# Autodesk Inventor assembly: MCOCWK26-6-12
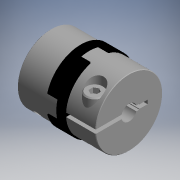
[picture p0: Inventor's stored thumbnail of the model, 180x180]
Saved by Autodesk Inventor 2017.3 (Build 213256000, 256)
## iProperties
Category: PARTsolutions
Company: MISUMI
Part Number: MCOCWK26-6-12
Catalog Web Link: www.cadenas.de
Description: MCOCLK, MCOCRK, MCOCWK-Oldham Clamping Type - Key Groove Hole Type
Vendor: MISUMI
Document SubType Name: Assembly
Designer: partserver
Manufacturer: MISUMI
Mass: 13.269 g
Surface Area: 80.443 cm^2
Volume: 13.269 cm^3
Density: 1 g/cm^3
Title: MCOCWK26-6-12
Author: Cadenas PARTsolutions
Comments: Oldham Clamping Type - Key Groove Hole Type
PSOL_IDENT_0: {$CADENAS_DATA\23d-libs\misumi\metric\50_couplings\mcocwk_asmtab.prj},243 {VTYP=3D},{STYP=ASSTAB},{N
PSOL_IDENT_1: B=MCOCWK26-6-12},{LINA=MCOCWK26-6-12},{NN=MCOCLK, MCOCRK, MCOCWK},{DATE=09.09.2019 15:28:19},{GEOMDA
PSOL_IDENT_2: TE=11.04.2017 04:14:27},{VERSION=},{LINEID=30},{WBVAR=KGHS,ALT1,LDC,DD1,ALT2,RDC,DD2,ALT3,ALT4},{WBN
PSOL_IDENT_3: UMERIC=LDC,RDC}  {NB=MCOCWK26-6-12},{LINA=MCOCWK26-6-12},{KT=DUMMY},{PN=MCOCWK26-6-12},{HS=},{KGHS=M
PSOL_IDENT_4: COCWK},{MATH=304 Stainless Steel Sintered Alloy},{MATS=Carbon Reinforced Resin},{AC=Hexagon Socket H
PSOL_IDENT_5: ead Cap Screw},{TYPE=MCOCWK},{NO=26},{D11='6','6','6.35','6.35','7','7','8','8','9.53','9.53','10','
PSOL_IDENT_6: 10','11','11','12','12'},{ALT1=},{ALT1ALG=},{DLALT1=6},{LDC=0.00},{LDCALG=0},{LDCALG1=},{LDCMIN=6},{
PSOL_IDENT_7: DD1=6},{DD1ALG1='6','6','6.35','6.35','7','7','8','8','9.53','9.53','10','10','11','11','12','12'},{
PSOL_IDENT_8: DD1ALG2=6},{D22='6','6','6.35','6.35','7','7','8','8','9.53','9.53','10','10','11','11','12','12'},{
PSOL_IDENT_9: ALT2=},{ALT2ALG=},{RDC=0.00},{RDCALG=[0]},{RDCALG1=},{DD2=12},{DD2ALG1='6','6','6.35','6.35','7','7'
PSOL_IDENT_10: ,'8','8','9.53','9.53','10','10','11','11','12','12'},{DD2ALG11='6','6','6.35','6.35','7','7','8','8'
PSOL_IDENT_11: ,'10','10','12','12'},{DD2ALG2=12},{DL=6},{DR=12},{D=26},{D1=27},{D2=29},{DD3=12.0},{L=30.4},{LL=11.
PSOL_IDENT_12: 5},{A=8.4},{A2=8.4},{F=5},{M=M4},{M2=M4},{T=3.0},{T2=3.0},{ALTALG2='','Select RDC'},{HSALG='MCOC','S
PSOL_IDENT_13: tandard Hole','','Key Groove Hole'},{KGHSALG='MCOCLK','d1 (One Side)','MCOCRK','d2 (One Side)','MCOC
PSOL_IDENT_14: WK','d1*d2 (Both Sides)'},{BBL=2},{TTL=1},{DD1NUM=6.000},{TTR=1.8},{DD2NUM=12},{BBR=4},{HSL=},{HSR=}
PSOL_IDENT_15: ,{DIA1=6},{DIA2=12},{ALT3=},{ALT3ALG= '', 'Not applicable'},{ALT3ALGPN=},{ALT4=},{ALT4ALG= '', 'w/o
PSOL_IDENT_16: KRH (Key Groove Width Change Right Shaft)', 'KRH' , 'with KRH (Key Groove Width Change Right Shaft)'
PSOL_IDENT_17: },{ALT4ALGPN=},{KLH=0},{KRH=5},{TTKLH=0.0},{TTKRH=2.3},{PPATH=mcoc/mcoc_asmtpl.prj}
NB: MCOCWK26-6-12
NN: MCOCLK, MCOCRK, MCOCWK
NT: Oldham Clamping Type - Key Groove Hole Type
NBSYN: $PN.
LINA: MCOCWK26-6-12
CATALOG: Misumi
PN: MCOCWK26-6-12
KGHS: d1*d2 (Both Sides)
MATH: 304 Stainless Steel Sintered Alloy
MATS: Carbon Reinforced Resin
AC: Hexagon Socket Head Cap Screw
NO: 26
ALT1: w/o LDC (Shaft Hole Diameter Left Shaft)
LDC: 0
DD1: 6
ALT2: w/o RDC (Shaft Hole Diameter Right Shaft)
RDC: 0
DD2: 12
D: 26
D1: 27
D2: 29
DD3: 12.0
L: 30.4
LL: 11.5
A: 8.4
A2: 8.4
F: 5
M: M4
M2: M4
T: 3.0
T2: 3.0
ALT3: Not applicable
ALT4: w/o KRH (Key Groove Width Change Right Shaft)
SUPPLIER: MISUMI
ARTICLENO: MCOCWK26-6-12
BOMINFO: MCOCWK26-6-12
CREATOR: CADENAS GmbH
## Documents named in this file (5)
- e:\temp\worker_35\temp\exporttempdir_1804_56_jDtGt\format_0\MCOCWK26-6-12.iam
- e:\temp\worker_35\temp\exporttempdir_1804_56_jDtGt\format_0\MCOC_spacer26.ipt
- e:\temp\worker_35\temp\exporttempdir_1804_56_jDtGt\format_0\MCOCWK26-6_c.ipt
- e:\temp\worker_35\temp\exporttempdir_1804_56_jDtGt\format_0\M4-12_bo2.ipt
- e:\temp\worker_35\temp\exporttempdir_1804_56_jDtGt\format_0\MCOCWK26-12_c.ipt
## Components (5 placed, 4 different names)
1. MCOC_spacer26:1 — C_XY@1 <-> L_XY@2, C_Z@1 <-> L_Z@2, C_YZ@1 <-> L_YZ@2, C_XY@1 <-> L_XY@4, C_Z@1 <-> L_Z@4, C_YZ@1 <-> L_YZ@4
2. MCOCWK26-6_c:1 — C_XY@1 <-> L_XY@2, C_Z@1 <-> L_Z@2, C_YZ@1 <-> L_YZ@2, screw_Z@2 <-> SCW_Z@3
3. M4-12_bo2:1 — screw_Z@2 <-> SCW_Z@3
4. MCOCWK26-12_c:1 — C_XY@1 <-> L_XY@4, C_Z@1 <-> L_Z@4, C_YZ@1 <-> L_YZ@4, screw_Z@4 <-> SCW_Z@5
5. M4-12_bo2:2 — screw_Z@4 <-> SCW_Z@5
## Relationships (8: Mate 5, Angle 2, Flush 1)
- C_XY@1 <-> L_XY@2 [Flush]: MCOC_spacer26:1 ↔ MCOCWK26-6_c:1
- C_Z@1 <-> L_Z@2 [Mate]: MCOC_spacer26:1 ↔ MCOCWK26-6_c:1
- C_YZ@1 <-> L_YZ@2 [Angle] (0 deg): MCOC_spacer26:1 ↔ MCOCWK26-6_c:1
- screw_Z@2 <-> SCW_Z@3 [Mate]: MCOCWK26-6_c:1 ↔ M4-12_bo2:1
- C_XY@1 <-> L_XY@4 [Mate]: MCOC_spacer26:1 ↔ MCOCWK26-12_c:1
- C_Z@1 <-> L_Z@4 [Mate]: MCOC_spacer26:1 ↔ MCOCWK26-12_c:1
- C_YZ@1 <-> L_YZ@4 [Angle] (90 deg): MCOC_spacer26:1 ↔ MCOCWK26-12_c:1
- screw_Z@4 <-> SCW_Z@5 [Mate]: MCOCWK26-12_c:1 ↔ M4-12_bo2:2
